# Autodesk Inventor assembly: assembled-feed
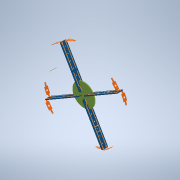
[picture p0: Inventor's stored thumbnail of the model, 180x180]
Saved by Autodesk Inventor 2021 (Build 250183000, 183)
## iProperties
Created: 2020-09-03
Part Number: assembled-feed
Document SubType Name: Assembly
Designer: dsouthall
Author: dsouthall
## Documents named in this file (3)
- C:\Users\dsouthall\OneDrive - The University of Chicago\Hpol\hpol-prototype\design\Quad-Slot\Model 8 in\assembled-feed.iam
- C:\Users\dsouthall\OneDrive - The University of Chicago\Hpol\hpol-prototype\design\Quad-Slot\Model 8 in\assembled-feed_feedline_8in.iam
- C:\Users\dsouthall\OneDrive - The University of Chicago\Hpol\hpol-prototype\design\Quad-Slot\Model 8 in\source\standin_quad_hub.ipt
## Components (5 placed, 2 different names)
1. assembled-feed_feedline_8in:1 [sub-assembly] — Mate:12, Mate:13, Mate:14
2. assembled-feed_feedline_8in:2 [sub-assembly] — Mate:9, Mate:10, Mate:11, Mate:15
3. assembled-feed_feedline_8in:3 [sub-assembly] — Mate:6, Mate:7, Mate:8, Mate:16
4. assembled-feed_feedline_8in:4 [sub-assembly] — Mate:3, Mate:4, Mate:5, Mate:17
5. standin_quad_hub:1 — Mate:1, Mate:2, Mate:3, Mate:4, Mate:5, Mate:6, Mate:7, Mate:8, Mate:9, Mate:10, Mate:11, Mate:12, Mate:13, Mate:14, Mate:15, Mate:16, Mate:17
## Relationships (18: Mate 17, Flush 1)
- Flush:1 (-3.9973 mm)
- Mate:1: standin_quad_hub:1
- Mate:2: standin_quad_hub:1
- Mate:3: assembled-feed_feedline_8in:4 ↔ standin_quad_hub:1
- Mate:4: assembled-feed_feedline_8in:4 ↔ standin_quad_hub:1
- Mate:5: assembled-feed_feedline_8in:4 ↔ standin_quad_hub:1
- Mate:6: assembled-feed_feedline_8in:3 ↔ standin_quad_hub:1
- Mate:7: assembled-feed_feedline_8in:3 ↔ standin_quad_hub:1
- Mate:8: assembled-feed_feedline_8in:3 ↔ standin_quad_hub:1
- Mate:9: assembled-feed_feedline_8in:2 ↔ standin_quad_hub:1
- Mate:10: assembled-feed_feedline_8in:2 ↔ standin_quad_hub:1
- Mate:11: assembled-feed_feedline_8in:2 ↔ standin_quad_hub:1
- Mate:12: assembled-feed_feedline_8in:1 ↔ standin_quad_hub:1
- Mate:13: assembled-feed_feedline_8in:1 ↔ standin_quad_hub:1
- Mate:14: assembled-feed_feedline_8in:1 ↔ standin_quad_hub:1
- Mate:15: assembled-feed_feedline_8in:2 ↔ standin_quad_hub:1
- Mate:16: assembled-feed_feedline_8in:3 ↔ standin_quad_hub:1
- Mate:17: assembled-feed_feedline_8in:4 ↔ standin_quad_hub:1
